# Autodesk Inventor assembly: X_Carriage_V2_0
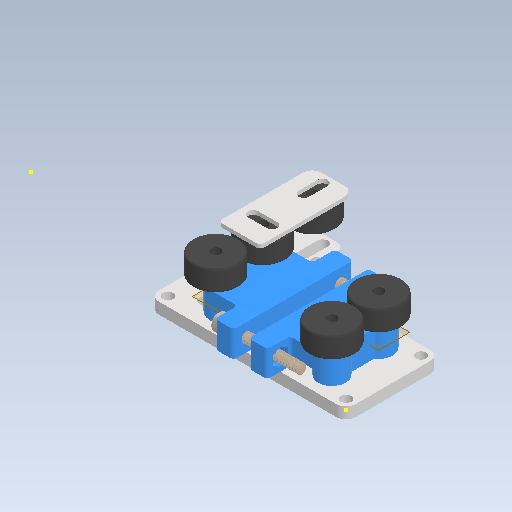
[picture p0: Inventor's stored thumbnail of the model, 512x512]
Saved by Autodesk Inventor 2021 (Build 250183000, 183)
## iProperties
Created: 2021-06-13
Part Number: X_Carriage_V2_0
Document SubType Name: Assembly
Designer: Jorian Brusind
Author: Jorian Brusind
## Documents named in this file (6)
- C:\Users\Jorian Brusind\Documents\GitHub\PersonalProjects\HyperRail\Inventor Files\X_Carriage_V2_0.iam
- C:\Users\Jorian Brusind\Documents\GitHub\PersonalProjects\HyperRail\Inventor Files\X_Carriage_Plate.ipt
- C:\Users\Jorian Brusind\Documents\GitHub\PersonalProjects\HyperRail\Inventor Files\11mm_BearingWheel.ipt
- C:\Users\Jorian Brusind\Documents\GitHub\PersonalProjects\HyperRail\Inventor Files\Belt_Restraint.ipt
- C:\Users\Jorian Brusind\Documents\GitHub\PersonalProjects\HyperRail\Inventor Files\4mm_Roller_Spacer.ipt
- C:\Users\Jorian Brusind\Documents\GitHub\PersonalProjects\Inventor Projects\Useful models\Metric bolt\Bolt M5 40mm.ipt
## Components (11 placed, 5 different names)
1. X_Carriage_Plate:1 — Mate:1, Mate:2, Mate:3, Mate:5, Mate:7, Mate:8, Mate:9, Mate:10, Flush:4, Mate:12, Mate:13, Mate:14, Mate:17
2. 11mm_BearingWheel:1 — Mate:1, Mate:6, Flush:2, Mate:15
3. 11mm_BearingWheel:2 — Mate:5, Mate:6, Flush:1, Mate:11
4. 11mm_BearingWheel:3 — Mate:3, Mate:4, Flush:1, Flush:3
5. 11mm_BearingWheel:4 — Mate:2, Mate:4, Flush:2, Flush:3, Mate:7, Mate:16
6. 11mm_BearingWheel:5 — Mate:8, Mate:9, Mate:10
7. Belt_Restraint:1 — Flush:4, Mate:11
8. 4mm_Roller_Spacer:1 — Mate:12, Mate:13, Mate:14, Mate:18, Mate:20, Mate:21
9. 4mm_Roller_Spacer:2 — Mate:15, Mate:16, Mate:17, Mate:19
10. Bolt M5 40mm:1 — Mate:19, Mate:21
11. Bolt M5 40mm:2 — Mate:18, Mate:20
## Relationships (25: Mate 21, Flush 4)
- Mate:1: X_Carriage_Plate:1 ↔ 11mm_BearingWheel:1
- Mate:2: X_Carriage_Plate:1 ↔ 11mm_BearingWheel:4
- Mate:3 (2.75 mm): X_Carriage_Plate:1 ↔ 11mm_BearingWheel:3
- Mate:4 (62 mm): 11mm_BearingWheel:3 ↔ 11mm_BearingWheel:4
- Mate:5 (2.75 mm): X_Carriage_Plate:1 ↔ 11mm_BearingWheel:2
- Mate:6 (62 mm): 11mm_BearingWheel:1 ↔ 11mm_BearingWheel:2
- Flush:1: 11mm_BearingWheel:2 ↔ 11mm_BearingWheel:3
- Flush:2: 11mm_BearingWheel:1 ↔ 11mm_BearingWheel:4
- Flush:3: 11mm_BearingWheel:3 ↔ 11mm_BearingWheel:4
- Mate:7 (15 mm): X_Carriage_Plate:1 ↔ 11mm_BearingWheel:4
- Mate:8 (2.75 mm): X_Carriage_Plate:1 ↔ 11mm_BearingWheel:5
- Mate:9 (-10 mm): X_Carriage_Plate:1 ↔ 11mm_BearingWheel:5
- Mate:10 (15 mm): X_Carriage_Plate:1 ↔ 11mm_BearingWheel:5
- Flush:4 (12 mm): X_Carriage_Plate:1 ↔ Belt_Restraint:1
- Mate:11: 11mm_BearingWheel:2 ↔ Belt_Restraint:1
- Mate:12: X_Carriage_Plate:1 ↔ 4mm_Roller_Spacer:1
- Mate:13: X_Carriage_Plate:1 ↔ 4mm_Roller_Spacer:1
- Mate:14: X_Carriage_Plate:1 ↔ 4mm_Roller_Spacer:1
- Mate:15: 11mm_BearingWheel:1 ↔ 4mm_Roller_Spacer:2
- Mate:16: 11mm_BearingWheel:4 ↔ 4mm_Roller_Spacer:2
- Mate:17: X_Carriage_Plate:1 ↔ 4mm_Roller_Spacer:2
- Mate:18: 4mm_Roller_Spacer:1 ↔ Bolt M5 40mm:2
- Mate:19: 4mm_Roller_Spacer:2 ↔ Bolt M5 40mm:1
- Mate:20: 4mm_Roller_Spacer:1 ↔ Bolt M5 40mm:2
- Mate:21: 4mm_Roller_Spacer:1 ↔ Bolt M5 40mm:1
